# Autodesk Inventor assembly: Shoulder
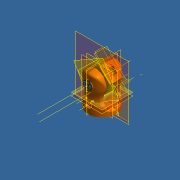
[picture p0: Inventor's stored thumbnail of the model, 180x180]
Saved by Autodesk Inventor 2016 (Build 200138000, 138)
## iProperties
Created: 2015-01-06
Part Number: Shoulder
Document SubType Name: Assembly
Designer: 4ndreas
Author: 4ndreas
## Documents named in this file (26)
- C:\Users\4ndreas\Documents\Inventor\RobotARM v2\v3\Shoulder.iam
- C:\Users\4ndreas\Documents\Inventor\RobotARM v2\v2\BaseJoint\Konstruktions-Assistent\Übertragung des Zahnriemens1.iam
- C:\Users\4ndreas\Documents\Inventor\RobotARM v2\v2\banebots_P6_3_stages.ipt
- C:\Users\4ndreas\Documents\Inventor\RobotARM v2\v2\Joint_A.ipt
- C:\Users\4ndreas\Documents\Inventor\RobotARM v2\v2\MotorKappe.ipt
- C:\Users\4ndreas\Documents\Inventor\Content Center Files\R2014\de-DE\DIN 931-1\DIN 931-1 - M8 x 60.ipt
- C:\Users\4ndreas\Documents\Inventor\Content Center Files\R2014\de-DE\DIN 625 - T1\DIN 625 T1 - 608 - 8 x 22 x 7.ipt
- C:\Users\4ndreas\Documents\Inventor\Content Center Files\R2014\de-DE\DIN 985\DIN 985 - M8.ipt
- C:\Users\4ndreas\Documents\Inventor\RobotARM v2\v2\Joint_A_gear_cut.ipt
- C:\Users\4ndreas\Documents\Inventor\RobotARM v2\v2\Nutplacer.ipt
- C:\Users\4ndreas\Documents\Inventor\Content Center Files\R2014\Leufter_30mm.ipt
- C:\Users\4ndreas\Documents\Inventor\Content Center Files\R2014\de-DE\ANSI B18.6.3(29)\ANSI B18.6.3 - 10-24 UNC - 0,5(13)135.ipt
- C:\Users\4ndreas\Documents\Inventor\Content Center Files\R2014\de-DE\DIN 125-1  A\DIN 125 - A 4,3.ipt
- C:\Users\4ndreas\Documents\Inventor\Content Center Files\R2014\de-DE\DIN BEARING(1)\DIN 625 SKF - SKF 624.ipt
- C:\Users\4ndreas\Documents\Inventor\Content Center Files\R2014\de-DE\DIN 433-1  A\DIN 433 - 4,3.ipt
- C:\Users\4ndreas\Documents\Inventor\RobotARM v2\v3\Shouder_spanner_Scheibe.ipt
- C:\Users\4ndreas\Documents\Inventor\RobotARM v2\v3\Shoulder_spanner.ipt
- C:\Users\4ndreas\Documents\Inventor\Content Center Files\R2014\de-DE\DIN 934\DIN 934 - M4 x 0,7.ipt
- C:\Users\4ndreas\Documents\Inventor\RobotARM v2\Nema17_GearedStepper.ipt
- C:\Users\4ndreas\Documents\Inventor\RobotARM v2\v3\Shoulder_bearing.ipt
- C:\Users\4ndreas\Documents\Inventor\RobotARM v2\v2\magHexMount.ipt
- C:\Users\4ndreas\Documents\Inventor\RobotARM v2\v2\encoder.iam
- C:\Users\4ndreas\Documents\Inventor\RobotARM v2\v3\Shoulder_stepper_holder.ipt
- C:\Users\4ndreas\Documents\Inventor\Content Center Files\R2014\de-DE\DIN 912\DIN 912 - M4 x 0,7 x 35 x 20.ipt
- C:\Users\4ndreas\Documents\Inventor\RobotARM v2\RotaryBase_r1.ipt
- C:\Users\4ndreas\Documents\Inventor\RobotARM v2\v3\Shoulder_deckplate.ipt
## Components (44 placed, 25 different names)
1. Shoulder_bearing:1 — Winkel:1, Passend:2, Passend:3, Fluchtend:1, Winkel:2, Passend:21, Passend:22, Passend:68, Passend:92, Passend:106, Winkel:9, Fluchtend:7, Passend:109, Passend:110, Passend:111, Passend:113, Passend:114, Passend:117, Passend:118, Passend:122, Passend:123, Passend:124, Passend:125
2. Übertragung des Zahnriemens:1 [sub-assembly] — Passend:5, Passend:7, Passend:1, Passend:12, Passend:19, Passend:29, Passend:49, Passend:69, Passend:72, Passend:94, Passend:95, Passend:107, Passend:112, Passend:115
3. banebots_P6_3_stages:1 — Passend:5, Passend:6, Passend:7, Passend:60, Passend:61, Passend:64, Passend:65, Passend:66, Passend:67, Passend:93, Fluchtend:8
4. Joint_A:1 — Passend:8, Passend:9, Passend:10, Fluchtend:2, Passend:11, Winkel:3, Passend:30
5. Joint_A_gear_cut:1 — Passend:9, Passend:10, Fluchtend:2, Passend:24, Winkel:5, Passend:40, Passend:41, Fluchtend:10
6. MotorKappe:1 — Winkel:8, Passend:50, Passend:125
7. DIN 931-1 - ersetzt durch DIN EN 24014 M8 x 60:1 — Passend:17, Passend:18, Passend:19, Passend:20, Passend:23, Passend:108
8. DIN 625 - T1 608 - 8 x 22 x 7:1 — Passend:17, Passend:22
9. DIN 625 - T1 608 - 8 x 22 x 7:2 — Passend:18, Passend:20, Passend:21
10. DIN 985 - ersetzt durch DIN EN ISO 10511 M8:1 — Passend:23, Passend:24, Winkel:5, Winkel:6
11. DIN 931-1 - ersetzt durch DIN EN 24014 M8 x 60:2 — Passend:25, Passend:26, Passend:27, Passend:28, Passend:29
12. DIN 625 - T1 608 - 8 x 22 x 7:3 — Passend:25, Passend:110
13. DIN 625 - T1 608 - 8 x 22 x 7:4 — Passend:26, Passend:27, Passend:111
14. DIN 985 - ersetzt durch DIN EN ISO 10511 M8:2 — Passend:28, Winkel:6, Passend:30
15. Shoulder_deckplate:1 — Passend:40, Passend:41, Fluchtend:10
16. Nutplacer:1
17. Leufter_30mm:1 — Passend:48, Winkel:8, Passend:50
18. Flachrundkopfschraube mit Kreuzschlitz - Typ II - Zoll Nr. 10 - 24 - 1/2:2 — Passend:65, Fluchtend:4
19. Flachrundkopfschraube mit Kreuzschlitz - Typ II - Zoll Nr. 10 - 24 - 1/2:1 — Passend:64, Fluchtend:4, Fluchtend:6, Passend:68
20. Flachrundkopfschraube mit Kreuzschlitz - Typ II - Zoll Nr. 10 - 24 - 1/2:3 — Passend:67, Fluchtend:5
21. Flachrundkopfschraube mit Kreuzschlitz - Typ II - Zoll Nr. 10 - 24 - 1/2:4 — Passend:66, Fluchtend:5, Fluchtend:6
22. DIN 912 - ersetzt durch DIN EN ISO 4762 M4 x 35:2 — Passend:70, Passend:71, Passend:72, Passend:77, Passend:78, Passend:87, Passend:88, Passend:91, Passend:97
23. DIN 912 - ersetzt durch DIN EN ISO 4762 M4 x 35:1 — Passend:69, Passend:73, Passend:74, Passend:82, Passend:83, Passend:85, Passend:99, Passend:104
24. DIN 125-1 A A 4,3:1 — Passend:70, Passend:71, Fluchtend:9
25. DIN 125-1 A A 4,3:2 — Passend:73, Passend:74, Passend:109, Fluchtend:9
26. DIN 625 SKF 624:1 — Passend:78, Passend:79, Passend:90
27. DIN 625 SKF 624:2 — Passend:77, Passend:79, Passend:89
28. DIN 625 SKF 624:3 — Passend:80, Passend:81, Passend:82, Passend:84
29. DIN 625 SKF 624:4 — Passend:80, Passend:81, Passend:86
30. DIN 433-1 A 4,3:1 — Passend:87, Passend:90, Passend:103
31. DIN 433-1 A 4,3:2 — Passend:83, Passend:84
32. DIN 433-1 A 4,3:3 — Passend:85, Passend:86, Passend:105
33. DIN 433-1 A 4,3:4 — Passend:88, Passend:89
34. Shoulder_spanner:1 — Passend:93, Passend:94, Passend:95, Passend:96, Passend:98, Passend:100, Passend:101, Passend:102
35. Shouder_spanner_Scheibe:2 — Passend:91, Passend:92, Passend:103
36. DIN 934 - ersetzt durch DIN EN 24032/28673/28674 M4:1 — Passend:99, Passend:100, Passend:101
37. DIN 934 - ersetzt durch DIN EN 24032/28673/28674 M4:2 — Passend:97, Passend:98, Passend:102
38. Shouder_spanner_Scheibe:3 — Passend:104, Passend:105, Passend:106
39. Nema17_GearedStepper:1 — Passend:107, Winkel:9, Fluchtend:8
40. magHexMount:1 — Passend:108, Passend:115
41. encoder:1 [sub-assembly] — Passend:112, Passend:113, Passend:114
42. Shoulder_stepper_holder:1
43. encoder:2 [sub-assembly] — Passend:116, Passend:117, Passend:118
44. RotaryBase_r1:2 — Passend:122, Passend:123, Passend:124
## Relationships (108: Mate 92, Flush 9, Angle 7)
- Passend:1 [Mate]: Übertragung des Zahnriemens:1
- Winkel:1 [Angle] (180 deg): Shoulder_bearing:1
- Passend:2 [Mate]: Shoulder_bearing:1
- Passend:3 [Mate]: Shoulder_bearing:1
- Fluchtend:1 [Flush] (12 mm): Shoulder_bearing:1
- Passend:4 [Mate]
- Winkel:2 [Angle] (90 deg): Shoulder_bearing:1
- Passend:5 [Mate]: Übertragung des Zahnriemens:1 ↔ banebots_P6_3_stages:1
- Passend:6 [Mate]: banebots_P6_3_stages:1
- Passend:7 [Mate] (5 mm): Übertragung des Zahnriemens:1 ↔ banebots_P6_3_stages:1
- Passend:8 [Mate]: Joint_A:1
- Passend:9 [Mate]: Joint_A:1 ↔ Joint_A_gear_cut:1
- Passend:10 [Mate]: Joint_A:1 ↔ Joint_A_gear_cut:1
- Fluchtend:2 [Flush]: Joint_A:1 ↔ Joint_A_gear_cut:1
- Passend:11 [Mate]: Joint_A:1
- Winkel:3 [Angle] (0 deg): Joint_A:1
- Passend:12 [Mate]: Übertragung des Zahnriemens:1
- Passend:17 [Mate]: DIN 931-1 - ersetzt durch DIN EN 24014 M8 x 60:1 ↔ DIN 625 - T1 608 - 8 x 22 x 7:1
- Passend:18 [Mate]: DIN 931-1 - ersetzt durch DIN EN 24014 M8 x 60:1 ↔ DIN 625 - T1 608 - 8 x 22 x 7:2
- Passend:19 [Mate]: Übertragung des Zahnriemens:1 ↔ DIN 931-1 - ersetzt durch DIN EN 24014 M8 x 60:1
- Passend:20 [Mate]: DIN 931-1 - ersetzt durch DIN EN 24014 M8 x 60:1 ↔ DIN 625 - T1 608 - 8 x 22 x 7:2
- Passend:21 [Mate]: Shoulder_bearing:1 ↔ DIN 625 - T1 608 - 8 x 22 x 7:2
- Passend:22 [Mate]: Shoulder_bearing:1 ↔ DIN 625 - T1 608 - 8 x 22 x 7:1
- Passend:23 [Mate]: DIN 931-1 - ersetzt durch DIN EN 24014 M8 x 60:1 ↔ DIN 985 - ersetzt durch DIN EN ISO 10511 M8:1
- Passend:24 [Mate]: Joint_A_gear_cut:1 ↔ DIN 985 - ersetzt durch DIN EN ISO 10511 M8:1
- Winkel:5 [Angle] (0 deg): Joint_A_gear_cut:1 ↔ DIN 985 - ersetzt durch DIN EN ISO 10511 M8:1
- Passend:25 [Mate]: DIN 931-1 - ersetzt durch DIN EN 24014 M8 x 60:2 ↔ DIN 625 - T1 608 - 8 x 22 x 7:3
- Passend:26 [Mate]: DIN 931-1 - ersetzt durch DIN EN 24014 M8 x 60:2 ↔ DIN 625 - T1 608 - 8 x 22 x 7:4
- Passend:27 [Mate]: DIN 931-1 - ersetzt durch DIN EN 24014 M8 x 60:2 ↔ DIN 625 - T1 608 - 8 x 22 x 7:4
- Passend:28 [Mate]: DIN 931-1 - ersetzt durch DIN EN 24014 M8 x 60:2 ↔ DIN 985 - ersetzt durch DIN EN ISO 10511 M8:2
- Passend:29 [Mate]: Übertragung des Zahnriemens:1 ↔ DIN 931-1 - ersetzt durch DIN EN 24014 M8 x 60:2
- Winkel:6 [Angle] (0 deg): DIN 985 - ersetzt durch DIN EN ISO 10511 M8:1 ↔ DIN 985 - ersetzt durch DIN EN ISO 10511 M8:2
- Passend:30 [Mate]: Joint_A:1 ↔ DIN 985 - ersetzt durch DIN EN ISO 10511 M8:2
- Passend:40 [Mate]: Joint_A_gear_cut:1 ↔ Shoulder_deckplate:1
- Passend:41 [Mate]: Joint_A_gear_cut:1 ↔ Shoulder_deckplate:1
- Passend:48 [Mate]: Leufter_30mm:1
- Passend:49 [Mate]: Übertragung des Zahnriemens:1
- Winkel:8 [Angle] (0 deg): MotorKappe:1 ↔ Leufter_30mm:1
- Passend:50 [Mate]: MotorKappe:1 ↔ Leufter_30mm:1
- Passend:60 [Mate]: banebots_P6_3_stages:1
- Passend:61 [Mate]: banebots_P6_3_stages:1
- Passend:62 [Mate]
- Passend:63 [Mate]
- Passend:64 [Mate]: banebots_P6_3_stages:1 ↔ Flachrundkopfschraube mit Kreuzschlitz - Typ II - Zoll Nr. 10 - 24 - 1/2:1
- Passend:65 [Mate]: banebots_P6_3_stages:1 ↔ Flachrundkopfschraube mit Kreuzschlitz - Typ II - Zoll Nr. 10 - 24 - 1/2:2
- Passend:66 [Mate]: banebots_P6_3_stages:1 ↔ Flachrundkopfschraube mit Kreuzschlitz - Typ II - Zoll Nr. 10 - 24 - 1/2:4
- Passend:67 [Mate]: banebots_P6_3_stages:1 ↔ Flachrundkopfschraube mit Kreuzschlitz - Typ II - Zoll Nr. 10 - 24 - 1/2:3
- Fluchtend:4 [Flush]: Flachrundkopfschraube mit Kreuzschlitz - Typ II - Zoll Nr. 10 - 24 - 1/2:2 ↔ Flachrundkopfschraube mit Kreuzschlitz - Typ II - Zoll Nr. 10 - 24 - 1/2:1
- Fluchtend:5 [Flush]: Flachrundkopfschraube mit Kreuzschlitz - Typ II - Zoll Nr. 10 - 24 - 1/2:3 ↔ Flachrundkopfschraube mit Kreuzschlitz - Typ II - Zoll Nr. 10 - 24 - 1/2:4
- Fluchtend:6 [Flush]: Flachrundkopfschraube mit Kreuzschlitz - Typ II - Zoll Nr. 10 - 24 - 1/2:1 ↔ Flachrundkopfschraube mit Kreuzschlitz - Typ II - Zoll Nr. 10 - 24 - 1/2:4
- Passend:68 [Mate]: Shoulder_bearing:1 ↔ Flachrundkopfschraube mit Kreuzschlitz - Typ II - Zoll Nr. 10 - 24 - 1/2:1
- Passend:69 [Mate]: Übertragung des Zahnriemens:1 ↔ DIN 912 - ersetzt durch DIN EN ISO 4762 M4 x 35:1
- Passend:70 [Mate]: DIN 912 - ersetzt durch DIN EN ISO 4762 M4 x 35:2 ↔ DIN 125-1 A A 4,3:1
- Passend:71 [Mate]: DIN 912 - ersetzt durch DIN EN ISO 4762 M4 x 35:2 ↔ DIN 125-1 A A 4,3:1
- Passend:72 [Mate]: Übertragung des Zahnriemens:1 ↔ DIN 912 - ersetzt durch DIN EN ISO 4762 M4 x 35:2
- Passend:73 [Mate]: DIN 912 - ersetzt durch DIN EN ISO 4762 M4 x 35:1 ↔ DIN 125-1 A A 4,3:2
- Passend:74 [Mate]: DIN 912 - ersetzt durch DIN EN ISO 4762 M4 x 35:1 ↔ DIN 125-1 A A 4,3:2
- Passend:77 [Mate]: DIN 912 - ersetzt durch DIN EN ISO 4762 M4 x 35:2 ↔ DIN 625 SKF 624:2
- Passend:78 [Mate]: DIN 912 - ersetzt durch DIN EN ISO 4762 M4 x 35:2 ↔ DIN 625 SKF 624:1
- Passend:79 [Mate]: DIN 625 SKF 624:1 ↔ DIN 625 SKF 624:2
- Passend:80 [Mate]: DIN 625 SKF 624:3 ↔ DIN 625 SKF 624:4
- Passend:81 [Mate]: DIN 625 SKF 624:3 ↔ DIN 625 SKF 624:4
- Passend:82 [Mate]: DIN 912 - ersetzt durch DIN EN ISO 4762 M4 x 35:1 ↔ DIN 625 SKF 624:3
- Passend:83 [Mate]: DIN 912 - ersetzt durch DIN EN ISO 4762 M4 x 35:1 ↔ DIN 433-1 A 4,3:2
- Passend:84 [Mate]: DIN 625 SKF 624:3 ↔ DIN 433-1 A 4,3:2
- Passend:85 [Mate]: DIN 912 - ersetzt durch DIN EN ISO 4762 M4 x 35:1 ↔ DIN 433-1 A 4,3:3
- Passend:86 [Mate]: DIN 625 SKF 624:4 ↔ DIN 433-1 A 4,3:3
- Passend:87 [Mate]: DIN 912 - ersetzt durch DIN EN ISO 4762 M4 x 35:2 ↔ DIN 433-1 A 4,3:1
- Passend:88 [Mate]: DIN 912 - ersetzt durch DIN EN ISO 4762 M4 x 35:2 ↔ DIN 433-1 A 4,3:4
- Passend:89 [Mate]: DIN 625 SKF 624:2 ↔ DIN 433-1 A 4,3:4
- Passend:90 [Mate]: DIN 625 SKF 624:1 ↔ DIN 433-1 A 4,3:1
- Passend:91 [Mate]: DIN 912 - ersetzt durch DIN EN ISO 4762 M4 x 35:2 ↔ Shouder_spanner_Scheibe:2
- Passend:92 [Mate]: Shoulder_bearing:1 ↔ Shouder_spanner_Scheibe:2
- Passend:93 [Mate]: banebots_P6_3_stages:1 ↔ Shoulder_spanner:1
- Passend:94 [Mate]: Übertragung des Zahnriemens:1 ↔ Shoulder_spanner:1
- Passend:95 [Mate]: Übertragung des Zahnriemens:1 ↔ Shoulder_spanner:1
- Passend:96 [Mate]: Shoulder_spanner:1
- Passend:97 [Mate]: DIN 912 - ersetzt durch DIN EN ISO 4762 M4 x 35:2 ↔ DIN 934 - ersetzt durch DIN EN 24032/28673/28674 M4:2
- Passend:98 [Mate]: Shoulder_spanner:1 ↔ DIN 934 - ersetzt durch DIN EN 24032/28673/28674 M4:2
- Passend:99 [Mate]: DIN 912 - ersetzt durch DIN EN ISO 4762 M4 x 35:1 ↔ DIN 934 - ersetzt durch DIN EN 24032/28673/28674 M4:1
- Passend:100 [Mate]: Shoulder_spanner:1 ↔ DIN 934 - ersetzt durch DIN EN 24032/28673/28674 M4:1
- Passend:101 [Mate]: Shoulder_spanner:1 ↔ DIN 934 - ersetzt durch DIN EN 24032/28673/28674 M4:1
- Passend:102 [Mate]: Shoulder_spanner:1 ↔ DIN 934 - ersetzt durch DIN EN 24032/28673/28674 M4:2
- Passend:103 [Mate]: DIN 433-1 A 4,3:1 ↔ Shouder_spanner_Scheibe:2
- Passend:104 [Mate]: DIN 912 - ersetzt durch DIN EN ISO 4762 M4 x 35:1 ↔ Shouder_spanner_Scheibe:3
- Passend:105 [Mate]: DIN 433-1 A 4,3:3 ↔ Shouder_spanner_Scheibe:3
- Passend:106 [Mate]: Shoulder_bearing:1 ↔ Shouder_spanner_Scheibe:3
- Passend:107 [Mate]: Übertragung des Zahnriemens:1 ↔ Nema17_GearedStepper:1
- Winkel:9 [Angle] (0 deg): Shoulder_bearing:1 ↔ Nema17_GearedStepper:1
- Passend:108 [Mate] (1.5 mm): DIN 931-1 - ersetzt durch DIN EN 24014 M8 x 60:1 ↔ magHexMount:1
- Fluchtend:7 [Flush] (44 mm): Shoulder_bearing:1
- Fluchtend:8 [Flush]: banebots_P6_3_stages:1 ↔ Nema17_GearedStepper:1
- Passend:109 [Mate]: Shoulder_bearing:1 ↔ DIN 125-1 A A 4,3:2
- Fluchtend:9 [Flush]: DIN 125-1 A A 4,3:1 ↔ DIN 125-1 A A 4,3:2
- Passend:110 [Mate]: Shoulder_bearing:1 ↔ DIN 625 - T1 608 - 8 x 22 x 7:3
- Passend:111 [Mate]: Shoulder_bearing:1 ↔ DIN 625 - T1 608 - 8 x 22 x 7:4
- Passend:112 [Mate]: Übertragung des Zahnriemens:1 ↔ encoder:1
- Passend:113 [Mate]: Shoulder_bearing:1 ↔ encoder:1
- Passend:114 [Mate]: Shoulder_bearing:1 ↔ encoder:1
- Passend:115 [Mate]: Übertragung des Zahnriemens:1 ↔ magHexMount:1
- Passend:116 [Mate]: encoder:2
- Passend:117 [Mate]: Shoulder_bearing:1 ↔ encoder:2
- Passend:118 [Mate]: Shoulder_bearing:1 ↔ encoder:2
- Passend:122 [Mate]: Shoulder_bearing:1 ↔ RotaryBase_r1:2
- Passend:123 [Mate]: Shoulder_bearing:1 ↔ RotaryBase_r1:2
- Passend:124 [Mate]: Shoulder_bearing:1 ↔ RotaryBase_r1:2
- Fluchtend:10 [Flush]: Joint_A_gear_cut:1 ↔ Shoulder_deckplate:1
- Passend:125 [Mate]: Shoulder_bearing:1 ↔ MotorKappe:1
